# Autodesk Inventor assembly: All Structures Assembly
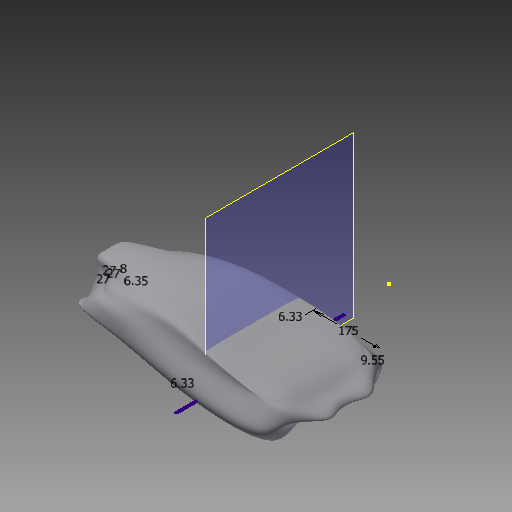
[picture p0: Inventor's stored thumbnail of the model, 512x512]
Saved by Autodesk Inventor 2018 (Build 220112000, 112)
## iProperties
Created: 2018-08-08
Part Number: All Structures Assembly
Document SubType Name: Assembly
Designer: Michael Gunderman
Author: Michael Gunderman
## Documents named in this file (2)
- C:\Users\Michael Gunderman\Documents\Special Projects\Echo 1\8-7-18\Echo-1-master\Echo 1\CAD work\Structures\All Structures Assembly.iam
- C:\Users\Michael Gunderman\Documents\Special Projects\Echo 1\8-7-18\Echo-1-master\Echo 1\CAD work\Structures\Fuselage\Fuselage Structure Assembly.iam
## Components (1 placed, 1 different names)
1. Fuselage Structure Assembly:1 [sub-assembly] — Flush:1, Flush:2, Flush:3
## Relationships (3: Flush 3)
- Flush:1: Fuselage Structure Assembly:1
- Flush:2: Fuselage Structure Assembly:1
- Flush:3: Fuselage Structure Assembly:1
